# Autodesk Inventor assembly: ARM_042_IntakeFULLAssemblyNewer
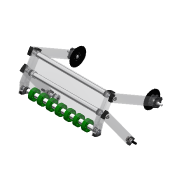
[picture p0: Inventor's stored thumbnail of the model, 180x180]
Saved by Autodesk Inventor 2018 (Build 220112000, 112)
## iProperties
Created: 2020-02-05
Part Number: ARM_042_IntakeFULLAssemblyNewer
Document SubType Name: Assembly
Designer: 22turnmaxw
Mass: 4854.19 g
Surface Area: 17228.7 cm^2
Volume: 2157.03 cm^3
Density: 2.25041 g/cm^3
Author: 22turnmaxw
## Documents named in this file (30)
- C:\Users\Myers.000\Documents\GrabCAD\Infinite Recharge 2020\Build season\ARM_042_IntakeFULLAssemblyNewer.iam
- C:\Users\Myers.000\Documents\GrabCAD\Infinite Recharge 2020\Build season\ARM_031_TwoPieceIntake.iam
- C:\Users\Myers.000\Documents\GrabCAD\Infinite Recharge 2020\Build season\ARM_032_3_OD_Straight_Flex_Wheel_217-6447.ipt
- C:\Users\Myers.000\Documents\GrabCAD\Infinite Recharge 2020\Build season\ARM_036_TopandBottomRollers.iam
- C:\Users\Myers.000\Documents\GrabCAD\Infinite Recharge 2020\Build season\ARM_072_SideBar13v2.ipt
- C:\Users\Myers.000\Documents\GrabCAD\Infinite Recharge 2020\Build season\ARM_071_SideBar15v2.ipt
- C:\Users\Myers.000\Documents\GrabCAD\Infinite Recharge 2020\Build season\ARM_039_MiddleRoller.iam
- C:\Users\Myers.000\Documents\GrabCAD\Infinite Recharge 2020\Build season\ARM_052_0.375ID_FlangedBearing.ipt
- C:\Users\Myers.000\Documents\GrabCAD\Infinite Recharge 2020\Build season\ARM_053_1.5inShoulderScrew.ipt
- C:\Users\Myers.000\Documents\GrabCAD\Infinite Recharge 2020\Build season\ARM_054_0.0625inSpacer.ipt
- C:\Users\Myers.000\Documents\GrabCAD\Infinite Recharge 2020\Build season\ARM_057_1.125inThunderHexBearing.ipt
- C:\Users\Myers.000\Documents\GrabCAD\Infinite Recharge 2020\Build season\ARM_058_BottomRoller.iam
- C:\Users\Myers.000\Documents\GrabCAD\Infinite Recharge 2020\Build season\_64t_Aluminum_Plate_Sprocket_25_Chain_1-1_8_Bearing_Bore_217-2629.ipt
- C:\Users\Myers.000\Documents\GrabCAD\Infinite Recharge 2020\Build season\VersaBlock_V2_217-6111_Combined.iam
- C:\Users\Myers.000\Documents\GrabCAD\Infinite Recharge 2020\Build season\ARM_060_1_125_Bearing_Pilot_Plastic_VersaHub_1_4_Wide_w_Plate_Sprocket_Mount_217-3234.ipt
- C:\Users\Myers.000\Documents\GrabCAD\Infinite Recharge 2020\Build season\ARM_062_4BarDrivingStubAxle.ipt
- C:\Users\Myers.000\Documents\GrabCAD\Infinite Recharge 2020\Build season\ARM_063_IntakeDrivingStubAxle.ipt
- C:\Users\Myers.000\Documents\GrabCAD\Infinite Recharge 2020\Build season\DGB STEP\217-2731_0_500_flanged_bearing.ipt
- C:\Users\Myers.000\Documents\GrabCAD\Infinite Recharge 2020\Build season\ARM_064_Bottom4BarPasiveStubAxle.ipt
- C:\Users\Myers.000\Documents\GrabCAD\Infinite Recharge 2020\Build season\ARM_078_LexanIntakeCover.ipt
- C:\Users\Myers.000\Documents\GrabCAD\Infinite Recharge 2020\Build season\ARM_079_GuiderHolder.ipt
- C:\Users\Myers.000\Documents\GrabCAD\Infinite Recharge 2020\Build season\ARM_077_IntakeBallGuide.ipt
- C:\Users\Myers.000\Documents\GrabCAD\Infinite Recharge 2020\Build season\ARM_083_BallGuideAttachment.ipt
- C:\Users\Myers.000\Documents\GrabCAD\Infinite Recharge 2020\Build season\ARM_082_BallGuideHardstop.ipt
- C:\Users\Myers.000\Documents\GrabCAD\Infinite Recharge 2020\Build season\ARM_034_36Tx9mm3mmPitchPulley.ipt
- C:\Users\Myers.000\Documents\GrabCAD\Infinite Recharge 2020\Build season\ARM_044_SDP_a_6a53-040df0908.ipt
- C:\Users\Myers.000\Documents\GrabCAD\Infinite Recharge 2020\Build season\ARM_084_0.3125Spacer.ipt
- C:\Users\Myers.000\Documents\GrabCAD\Infinite Recharge 2020\Build season\ARM_085_0.0625Spacer.ipt
- C:\Users\Myers.000\Documents\GrabCAD\Infinite Recharge 2020\Build season\ARM_086_1.1875Spacer.ipt
- C:\Users\Myers.000\Documents\GrabCAD\Infinite Recharge 2020\Build season\ARM_091_IntakeSideCap(WithCutout).ipt
## Components (80 placed, 29 different names)
1. ARM_031_TwoPieceIntake:1 [sub-assembly] — Flush:1, Flush:2, Mate:1, Mate:61, Mate:66, Mate:67, Mate:68, Mate:69, Mate:78, Mate:101, Mate:125, Insert:13, Mate:142, Mate:143, Mate:144, Mate:145, Mate:161, Mate:184, Mate:185, Mate:186, Mate:196, Mate:197, Mate:198, Flush:17, Mate:214, Flush:18
2. ARM_031_TwoPieceIntake:2 [sub-assembly] — Flush:1, Flush:2, Mate:1, Mate:63, Mate:64, Mate:65, Mate:70, Mate:73, Mate:74, Mate:76, Mate:77, Mate:83, Mate:84, Mate:91, Mate:92, Mate:110, Mate:111, Mate:113, Mate:114, Mate:115, Insert:6, Mate:187, Mate:188, Mate:189, Mate:199, Mate:200, Mate:201
3. ARM_032_3_OD_Straight_Flex_Wheel_217-6447:1 — Mate:20, Mate:21, Rotation:13, Rotation:14, Mate:155
4. ARM_032_3_OD_Straight_Flex_Wheel_217-6447:2 — Mate:24, Rotation:16, Mate:61, Mate:158
5. ARM_032_3_OD_Straight_Flex_Wheel_217-6447:3 — Mate:22, Mate:23, Mate:24, Rotation:15, Rotation:16, Mate:157
6. ARM_032_3_OD_Straight_Flex_Wheel_217-6447:5 — Mate:18, Rotation:11, Mate:152
7. ARM_032_3_OD_Straight_Flex_Wheel_217-6447:6 — Mate:19, Mate:20, Rotation:12, Rotation:13, Mate:154
8. ARM_032_3_OD_Straight_Flex_Wheel_217-6447:7 — Mate:18, Mate:19, Rotation:11, Rotation:12, Mate:153
9. ARM_032_3_OD_Straight_Flex_Wheel_217-6447:8 — Mate:21, Mate:22, Mate:23, Rotation:14, Rotation:15, Mate:156
10. ARM_036_TopandBottomRollers:2 [sub-assembly] — Mate:76, Mate:78
11. ARM_072_SideBar13v2:1 — Mate:42, Mate:62, Mate:63, Mate:65, Insert:2, Insert:10, Insert:12, Mate:193, Mate:194, Mate:195, Mate:205, Mate:206, Mate:207
12. ARM_072_SideBar13v2:2 — Mate:42, Mate:66, Mate:68, Mate:102, Mate:106, Mate:107, Insert:9, Insert:11, Mate:190, Mate:191, Mate:192, Mate:208, Mate:209, Mate:210
13. ARM_071_SideBar15v2:1 — Mate:43, Mate:60, Mate:64, Mate:70, Mate:85, Mate:86, Mate:129, Mate:131, Mate:132, Angle:1, Mate:202, Mate:203, Mate:204
14. ARM_071_SideBar15v2:2 — Mate:43, Mate:55, Mate:67, Mate:69, Mate:103, Mate:104, Mate:105, Mate:108, Mate:134, Angle:4, Mate:135, Mate:211, Mate:212, Mate:213
15. ARM_039_MiddleRoller:1 [sub-assembly] — Mate:73, Mate:74, Mate:77, Mate:112, Flush:5, Flush:16
16. ARM_052_0.375ID_FlangedBearing:1 — Mate:79, Mate:80, Mate:82, Mate:83, Mate:84
17. ARM_052_0.375ID_FlangedBearing:2 — Mate:81, Mate:82
18. ARM_052_0.375ID_FlangedBearing:3 — Mate:85, Mate:86, Insert:1
19. ARM_052_0.375ID_FlangedBearing:4 — Insert:2, Insert:3
20. ARM_052_0.375ID_FlangedBearing:5 — Mate:87, Mate:88, Mate:90, Mate:91, Mate:92
21. ARM_052_0.375ID_FlangedBearing:6 — Mate:89, Mate:90
22. ARM_052_0.375ID_FlangedBearing:7 — Mate:93, Mate:94, Mate:96
23. ARM_052_0.375ID_FlangedBearing:8 — Mate:95, Mate:96, Mate:103, Mate:104
24. ARM_052_0.375ID_FlangedBearing:9 — Mate:105, Mate:108, Insert:4
25. ARM_052_0.375ID_FlangedBearing:10 — Mate:97, Mate:100
26. ARM_052_0.375ID_FlangedBearing:11 — Mate:106, Mate:107, Insert:5
27. ARM_052_0.375ID_FlangedBearing:12 — Mate:98, Mate:99, Mate:100, Mate:101, Mate:102
28. ARM_053_1.5inShoulderScrew:1 — Insert:4
29. ARM_053_1.5inShoulderScrew:2 — Insert:5
30. ARM_053_1.5inShoulderScrew:3 — Insert:1
31. ARM_053_1.5inShoulderScrew:4 — Insert:3
32. ARM_054_0.0625inSpacer:1 — Mate:79, Mate:80, Mate:81
33. ARM_054_0.0625inSpacer:2 — Mate:87, Mate:88, Mate:89
34. ARM_054_0.0625inSpacer:3 — Mate:93, Mate:94, Mate:95
35. ARM_054_0.0625inSpacer:4 — Mate:97, Mate:98, Mate:99
36. ARM_057_1.125inThunderHexBearing:1 — Mate:110, Mate:111, Mate:116, Mate:117
37. ARM_057_1.125inThunderHexBearing:3 — Mate:114, Mate:115
38. ARM_057_1.125inThunderHexBearing:4 — Mate:112, Mate:113
39. ARM_058_BottomRoller:1 [sub-assembly] — Mate:116, Mate:117, Mate:152, Mate:153, Mate:154, Mate:155, Mate:156, Mate:157, Mate:158
40. ARM_057_1.125inThunderHexBearing:5 — Insert:6
41. ARM_057_1.125inThunderHexBearing:6 — Insert:13
42. ARM_057_1.125inThunderHexBearing:7 — Mate:125, Mate:161
43. _64t_Aluminum_Plate_Sprocket_25_Chain_1-1_8_Bearing_Bore_217-2629:1 — Mate:129, Angle:3, Mate:133, Flush:14
44. VersaBlock_V2_217-6111_Combined:1 [sub-assembly] — Mate:131, Mate:132, Angle:1, Insert:7, Angle:2, Mate:139, Mate:174, Mate:175
45. ARM_060_1_125_Bearing_Pilot_Plastic_VersaHub_1_4_Wide_w_Plate_Sprocket_Mount_217-3234:1 — Insert:7, Angle:2, Angle:3, Mate:133
46. VersaBlock_V2_217-6111_Combined:2 [sub-assembly] — Mate:134, Angle:4, Mate:135, Mate:136, Angle:5, Mate:138, Mate:172, Mate:173, Mate:181
47. ARM_060_1_125_Bearing_Pilot_Plastic_VersaHub_1_4_Wide_w_Plate_Sprocket_Mount_217-3234:2 — Angle:5, Angle:6, Mate:137, Mate:172, Mate:173
48. _64t_Aluminum_Plate_Sprocket_25_Chain_1-1_8_Bearing_Bore_217-2629:2 — Mate:136, Angle:6, Mate:137, Flush:15
49. ARM_062_4BarDrivingStubAxle:1 — Mate:138, Flush:15, Mate:180
50. ARM_062_4BarDrivingStubAxle:2 — Mate:139, Flush:14
51. ARM_063_IntakeDrivingStubAxle:2 — Flush:5, Mate:140, Mate:167
52. 217-2731_0_500_flanged_bearing:1 — Insert:9, Mate:141, Mate:179
53. 217-2731_0_500_flanged_bearing:2 — Insert:11, Flush:6
54. 217-2731_0_500_flanged_bearing:3 — Insert:10, Mate:140, Mate:182
55. 217-2731_0_500_flanged_bearing:4 — Insert:12, Mate:176, Mate:177
56. ARM_064_Bottom4BarPasiveStubAxle:1 — Mate:141, Flush:6, Mate:178
57. ARM_057_1.125inThunderHexBearing:9 — Mate:144, Mate:145
58. ARM_057_1.125inThunderHexBearing:10 — Mate:142, Mate:143
59. ARM_078_LexanIntakeCover:1 — Flush:17, Mate:214, Flush:18, Mate:215
60. ARM_079_GuiderHolder:1 — Mate:160, Flush:10, Mate:163, Mate:164, Mate:215
61. ARM_077_IntakeBallGuide:1 — Mate:160, Flush:10, Mate:162, Flush:11, Flush:12
62. ARM_083_BallGuideAttachment:1 — Mate:162, Flush:11, Flush:12, Flush:13
63. ARM_082_BallGuideHardstop:1 — Mate:163, Flush:13, Mate:164
64. ARM_034_36Tx9mm3mmPitchPulley:1 — Mate:165, Mate:166, Mate:183
65. ARM_044_SDP_a_6a53-040df0908:1 — Mate:165, Mate:166, Flush:16, Mate:167
66. ARM_085_0.0625Spacer:1 — Mate:174, Mate:175
67. ARM_085_0.0625Spacer:2 — Mate:180, Mate:181
68. ARM_084_0.3125Spacer:1 — Mate:176, Mate:177
69. ARM_084_0.3125Spacer:2 — Mate:178, Mate:179
70. ARM_086_1.1875Spacer:1 — Mate:182, Mate:183
71. ARM_091_IntakeSideCap(WithCutout):1 — Mate:184, Mate:185, Mate:186
72. ARM_091_IntakeSideCap(WithCutout):4 — Mate:187, Mate:188, Mate:189
73. ARM_091_IntakeSideCap(WithCutout):6 — Mate:190, Mate:191, Mate:192
74. ARM_091_IntakeSideCap(WithCutout):7 — Mate:193, Mate:194, Mate:195
75. ARM_091_IntakeSideCap(WithCutout):8 — Mate:196, Mate:197, Mate:198
76. ARM_091_IntakeSideCap(WithCutout):9 — Mate:211, Mate:212, Mate:213
77. ARM_091_IntakeSideCap(WithCutout):11 — Mate:199, Mate:200, Mate:201
78. ARM_091_IntakeSideCap(WithCutout):12 — Mate:202, Mate:203, Mate:204
79. ARM_091_IntakeSideCap(WithCutout):14 — Mate:208, Mate:209, Mate:210
80. ARM_091_IntakeSideCap(WithCutout):15 — Mate:205, Mate:206, Mate:207
## Relationships (178: Mate 141, Flush 13, Insert 12, RelateRotation 6, Angle 6)
- Flush:1: ARM_031_TwoPieceIntake:1 ↔ ARM_031_TwoPieceIntake:2
- Flush:2: ARM_031_TwoPieceIntake:1 ↔ ARM_031_TwoPieceIntake:2
- Mate:1 (552.45 mm): ARM_031_TwoPieceIntake:1 ↔ ARM_031_TwoPieceIntake:2
- Mate:18 (44.45 mm): ARM_032_3_OD_Straight_Flex_Wheel_217-6447:5 ↔ ARM_032_3_OD_Straight_Flex_Wheel_217-6447:7
- Mate:19 (44.45 mm): ARM_032_3_OD_Straight_Flex_Wheel_217-6447:6 ↔ ARM_032_3_OD_Straight_Flex_Wheel_217-6447:7
- Mate:20 (44.45 mm): ARM_032_3_OD_Straight_Flex_Wheel_217-6447:1 ↔ ARM_032_3_OD_Straight_Flex_Wheel_217-6447:6
- Mate:21 (44.45 mm): ARM_032_3_OD_Straight_Flex_Wheel_217-6447:1 ↔ ARM_032_3_OD_Straight_Flex_Wheel_217-6447:8
- Mate:22 (44.45 mm): ARM_032_3_OD_Straight_Flex_Wheel_217-6447:3 ↔ ARM_032_3_OD_Straight_Flex_Wheel_217-6447:8
- Mate:23 (44.45 mm): ARM_032_3_OD_Straight_Flex_Wheel_217-6447:3 ↔ ARM_032_3_OD_Straight_Flex_Wheel_217-6447:8
- Mate:24 (44.45 mm): ARM_032_3_OD_Straight_Flex_Wheel_217-6447:2 ↔ ARM_032_3_OD_Straight_Flex_Wheel_217-6447:3
- Rotation:11 [RelateRotation] (1 ul): ARM_032_3_OD_Straight_Flex_Wheel_217-6447:5 ↔ ARM_032_3_OD_Straight_Flex_Wheel_217-6447:7
- Rotation:12 [RelateRotation] (1 ul): ARM_032_3_OD_Straight_Flex_Wheel_217-6447:6 ↔ ARM_032_3_OD_Straight_Flex_Wheel_217-6447:7
- Rotation:13 [RelateRotation] (1 ul): ARM_032_3_OD_Straight_Flex_Wheel_217-6447:1 ↔ ARM_032_3_OD_Straight_Flex_Wheel_217-6447:6
- Rotation:14 [RelateRotation] (1 ul): ARM_032_3_OD_Straight_Flex_Wheel_217-6447:1 ↔ ARM_032_3_OD_Straight_Flex_Wheel_217-6447:8
- Rotation:15 [RelateRotation] (1 ul): ARM_032_3_OD_Straight_Flex_Wheel_217-6447:3 ↔ ARM_032_3_OD_Straight_Flex_Wheel_217-6447:8
- Rotation:16 [RelateRotation] (1 ul): ARM_032_3_OD_Straight_Flex_Wheel_217-6447:2 ↔ ARM_032_3_OD_Straight_Flex_Wheel_217-6447:3
- Mate:42: ARM_072_SideBar13v2:1 ↔ ARM_072_SideBar13v2:2
- Mate:43: ARM_071_SideBar15v2:1 ↔ ARM_071_SideBar15v2:2
- Mate:55 (135.8138 mm): ARM_071_SideBar15v2:2
- Mate:60 (124.4092 mm): ARM_071_SideBar15v2:1
- Mate:61 (50.8 mm): ARM_031_TwoPieceIntake:1 ↔ ARM_032_3_OD_Straight_Flex_Wheel_217-6447:2
- Mate:62: ARM_072_SideBar13v2:1
- Mate:63 (4.7625 mm): ARM_031_TwoPieceIntake:2 ↔ ARM_072_SideBar13v2:1
- Mate:64: ARM_031_TwoPieceIntake:2 ↔ ARM_071_SideBar15v2:1
- Mate:65: ARM_031_TwoPieceIntake:2 ↔ ARM_072_SideBar13v2:1
- Mate:66: ARM_031_TwoPieceIntake:1 ↔ ARM_072_SideBar13v2:2
- Mate:67: ARM_031_TwoPieceIntake:1 ↔ ARM_071_SideBar15v2:2
- Mate:68 (4.7625 mm): ARM_031_TwoPieceIntake:1 ↔ ARM_072_SideBar13v2:2
- Mate:69 (4.7625 mm): ARM_031_TwoPieceIntake:1 ↔ ARM_071_SideBar15v2:2
- Mate:70 (4.7625 mm): ARM_031_TwoPieceIntake:2 ↔ ARM_071_SideBar15v2:1
- Mate:73: ARM_031_TwoPieceIntake:2 ↔ ARM_039_MiddleRoller:1
- Mate:74: ARM_031_TwoPieceIntake:2 ↔ ARM_039_MiddleRoller:1
- Mate:76: ARM_031_TwoPieceIntake:2 ↔ ARM_036_TopandBottomRollers:2
- Mate:77 (1.5875 mm): ARM_031_TwoPieceIntake:2 ↔ ARM_039_MiddleRoller:1
- Mate:78 (1.5875 mm): ARM_031_TwoPieceIntake:1 ↔ ARM_036_TopandBottomRollers:2
- Mate:79: ARM_052_0.375ID_FlangedBearing:1 ↔ ARM_054_0.0625inSpacer:1
- Mate:80: ARM_052_0.375ID_FlangedBearing:1 ↔ ARM_054_0.0625inSpacer:1
- Mate:81: ARM_052_0.375ID_FlangedBearing:2 ↔ ARM_054_0.0625inSpacer:1
- Mate:82: ARM_052_0.375ID_FlangedBearing:1 ↔ ARM_052_0.375ID_FlangedBearing:2
- Mate:83: ARM_031_TwoPieceIntake:2 ↔ ARM_052_0.375ID_FlangedBearing:1
- Mate:84: ARM_031_TwoPieceIntake:2 ↔ ARM_052_0.375ID_FlangedBearing:1
- Mate:85: ARM_071_SideBar15v2:1 ↔ ARM_052_0.375ID_FlangedBearing:3
- Mate:86: ARM_071_SideBar15v2:1 ↔ ARM_052_0.375ID_FlangedBearing:3
- Insert:1: ARM_052_0.375ID_FlangedBearing:3 ↔ ARM_053_1.5inShoulderScrew:3
- Mate:87: ARM_052_0.375ID_FlangedBearing:5 ↔ ARM_054_0.0625inSpacer:2
- Mate:88: ARM_052_0.375ID_FlangedBearing:5 ↔ ARM_054_0.0625inSpacer:2
- Mate:89: ARM_052_0.375ID_FlangedBearing:6 ↔ ARM_054_0.0625inSpacer:2
- Mate:90: ARM_052_0.375ID_FlangedBearing:5 ↔ ARM_052_0.375ID_FlangedBearing:6
- Mate:91: ARM_031_TwoPieceIntake:2 ↔ ARM_052_0.375ID_FlangedBearing:5
- Mate:92: ARM_031_TwoPieceIntake:2 ↔ ARM_052_0.375ID_FlangedBearing:5
- Insert:2: ARM_072_SideBar13v2:1 ↔ ARM_052_0.375ID_FlangedBearing:4
- Insert:3: ARM_052_0.375ID_FlangedBearing:4 ↔ ARM_053_1.5inShoulderScrew:4
- Mate:93: ARM_052_0.375ID_FlangedBearing:7 ↔ ARM_054_0.0625inSpacer:3
- Mate:94: ARM_052_0.375ID_FlangedBearing:7 ↔ ARM_054_0.0625inSpacer:3
- Mate:95: ARM_052_0.375ID_FlangedBearing:8 ↔ ARM_054_0.0625inSpacer:3
- Mate:96: ARM_052_0.375ID_FlangedBearing:7 ↔ ARM_052_0.375ID_FlangedBearing:8
- Mate:97: ARM_052_0.375ID_FlangedBearing:10 ↔ ARM_054_0.0625inSpacer:4
- Mate:98: ARM_052_0.375ID_FlangedBearing:12 ↔ ARM_054_0.0625inSpacer:4
- Mate:99: ARM_052_0.375ID_FlangedBearing:12 ↔ ARM_054_0.0625inSpacer:4
- Mate:100: ARM_052_0.375ID_FlangedBearing:10 ↔ ARM_052_0.375ID_FlangedBearing:12
- Mate:101: ARM_031_TwoPieceIntake:1 ↔ ARM_052_0.375ID_FlangedBearing:12
- Mate:102: ARM_072_SideBar13v2:2 ↔ ARM_052_0.375ID_FlangedBearing:12
- Mate:103: ARM_071_SideBar15v2:2 ↔ ARM_052_0.375ID_FlangedBearing:8
- Mate:104: ARM_071_SideBar15v2:2 ↔ ARM_052_0.375ID_FlangedBearing:8
- Mate:105: ARM_071_SideBar15v2:2 ↔ ARM_052_0.375ID_FlangedBearing:9
- Mate:106: ARM_072_SideBar13v2:2 ↔ ARM_052_0.375ID_FlangedBearing:11
- Mate:107: ARM_072_SideBar13v2:2 ↔ ARM_052_0.375ID_FlangedBearing:11
- Mate:108: ARM_071_SideBar15v2:2 ↔ ARM_052_0.375ID_FlangedBearing:9
- Insert:4: ARM_052_0.375ID_FlangedBearing:9 ↔ ARM_053_1.5inShoulderScrew:1
- Insert:5: ARM_052_0.375ID_FlangedBearing:11 ↔ ARM_053_1.5inShoulderScrew:2
- Mate:110: ARM_031_TwoPieceIntake:2 ↔ ARM_057_1.125inThunderHexBearing:1
- Mate:111: ARM_031_TwoPieceIntake:2 ↔ ARM_057_1.125inThunderHexBearing:1
- Mate:112: ARM_039_MiddleRoller:1 ↔ ARM_057_1.125inThunderHexBearing:4
- Mate:113: ARM_031_TwoPieceIntake:2 ↔ ARM_057_1.125inThunderHexBearing:4
- Mate:114: ARM_031_TwoPieceIntake:2 ↔ ARM_057_1.125inThunderHexBearing:3
- Mate:115: ARM_031_TwoPieceIntake:2 ↔ ARM_057_1.125inThunderHexBearing:3
- Mate:116: ARM_057_1.125inThunderHexBearing:1 ↔ ARM_058_BottomRoller:1
- Mate:117: ARM_057_1.125inThunderHexBearing:1 ↔ ARM_058_BottomRoller:1
- Insert:6: ARM_031_TwoPieceIntake:2 ↔ ARM_057_1.125inThunderHexBearing:5
- Mate:125: ARM_031_TwoPieceIntake:1 ↔ ARM_057_1.125inThunderHexBearing:7
- Mate:129: ARM_071_SideBar15v2:1 ↔ _64t_Aluminum_Plate_Sprocket_25_Chain_1-1_8_Bearing_Bore_217-2629:1
- Mate:131: ARM_071_SideBar15v2:1 ↔ VersaBlock_V2_217-6111_Combined:1
- Mate:132: ARM_071_SideBar15v2:1 ↔ VersaBlock_V2_217-6111_Combined:1
- Angle:1 (0 deg): ARM_071_SideBar15v2:1 ↔ VersaBlock_V2_217-6111_Combined:1
- Insert:7: VersaBlock_V2_217-6111_Combined:1 ↔ ARM_060_1_125_Bearing_Pilot_Plastic_VersaHub_1_4_Wide_w_Plate_Sprocket_Mount_217-3234:1
- Angle:2 (0 deg): VersaBlock_V2_217-6111_Combined:1 ↔ ARM_060_1_125_Bearing_Pilot_Plastic_VersaHub_1_4_Wide_w_Plate_Sprocket_Mount_217-3234:1
- Angle:3 (0 deg): _64t_Aluminum_Plate_Sprocket_25_Chain_1-1_8_Bearing_Bore_217-2629:1 ↔ ARM_060_1_125_Bearing_Pilot_Plastic_VersaHub_1_4_Wide_w_Plate_Sprocket_Mount_217-3234:1
- Mate:133: _64t_Aluminum_Plate_Sprocket_25_Chain_1-1_8_Bearing_Bore_217-2629:1 ↔ ARM_060_1_125_Bearing_Pilot_Plastic_VersaHub_1_4_Wide_w_Plate_Sprocket_Mount_217-3234:1
- Mate:134: ARM_071_SideBar15v2:2 ↔ VersaBlock_V2_217-6111_Combined:2
- Angle:4 (0 deg): ARM_071_SideBar15v2:2 ↔ VersaBlock_V2_217-6111_Combined:2
- Mate:135: ARM_071_SideBar15v2:2 ↔ VersaBlock_V2_217-6111_Combined:2
- Mate:136: VersaBlock_V2_217-6111_Combined:2 ↔ _64t_Aluminum_Plate_Sprocket_25_Chain_1-1_8_Bearing_Bore_217-2629:2
- Angle:5 (0 deg): VersaBlock_V2_217-6111_Combined:2 ↔ ARM_060_1_125_Bearing_Pilot_Plastic_VersaHub_1_4_Wide_w_Plate_Sprocket_Mount_217-3234:2
- Angle:6 (0 deg): ARM_060_1_125_Bearing_Pilot_Plastic_VersaHub_1_4_Wide_w_Plate_Sprocket_Mount_217-3234:2 ↔ _64t_Aluminum_Plate_Sprocket_25_Chain_1-1_8_Bearing_Bore_217-2629:2
- Mate:137: ARM_060_1_125_Bearing_Pilot_Plastic_VersaHub_1_4_Wide_w_Plate_Sprocket_Mount_217-3234:2 ↔ _64t_Aluminum_Plate_Sprocket_25_Chain_1-1_8_Bearing_Bore_217-2629:2
- Mate:138: VersaBlock_V2_217-6111_Combined:2 ↔ ARM_062_4BarDrivingStubAxle:1
- Mate:139: VersaBlock_V2_217-6111_Combined:1 ↔ ARM_062_4BarDrivingStubAxle:2
- Insert:9: ARM_072_SideBar13v2:2 ↔ 217-2731_0_500_flanged_bearing:1
- Insert:10: ARM_072_SideBar13v2:1 ↔ 217-2731_0_500_flanged_bearing:3
- Insert:11: ARM_072_SideBar13v2:2 ↔ 217-2731_0_500_flanged_bearing:2
- Insert:12: ARM_072_SideBar13v2:1 ↔ 217-2731_0_500_flanged_bearing:4
- Insert:13: ARM_031_TwoPieceIntake:1 ↔ ARM_057_1.125inThunderHexBearing:6
- Flush:5: ARM_039_MiddleRoller:1 ↔ ARM_063_IntakeDrivingStubAxle:2
- Mate:140: ARM_063_IntakeDrivingStubAxle:2 ↔ 217-2731_0_500_flanged_bearing:3
- Mate:141: 217-2731_0_500_flanged_bearing:1 ↔ ARM_064_Bottom4BarPasiveStubAxle:1
- Flush:6: 217-2731_0_500_flanged_bearing:2 ↔ ARM_064_Bottom4BarPasiveStubAxle:1
- Mate:142: ARM_031_TwoPieceIntake:1 ↔ ARM_057_1.125inThunderHexBearing:10
- Mate:143: ARM_031_TwoPieceIntake:1 ↔ ARM_057_1.125inThunderHexBearing:10
- Mate:144: ARM_031_TwoPieceIntake:1 ↔ ARM_057_1.125inThunderHexBearing:9
- Mate:145: ARM_031_TwoPieceIntake:1 ↔ ARM_057_1.125inThunderHexBearing:9
- Mate:152: ARM_032_3_OD_Straight_Flex_Wheel_217-6447:5 ↔ ARM_058_BottomRoller:1
- Mate:153: ARM_032_3_OD_Straight_Flex_Wheel_217-6447:7 ↔ ARM_058_BottomRoller:1
- Mate:154: ARM_032_3_OD_Straight_Flex_Wheel_217-6447:6 ↔ ARM_058_BottomRoller:1
- Mate:155: ARM_032_3_OD_Straight_Flex_Wheel_217-6447:1 ↔ ARM_058_BottomRoller:1
- Mate:156: ARM_032_3_OD_Straight_Flex_Wheel_217-6447:8 ↔ ARM_058_BottomRoller:1
- Mate:157: ARM_032_3_OD_Straight_Flex_Wheel_217-6447:3 ↔ ARM_058_BottomRoller:1
- Mate:158: ARM_032_3_OD_Straight_Flex_Wheel_217-6447:2 ↔ ARM_058_BottomRoller:1
- Mate:160: ARM_079_GuiderHolder:1 ↔ ARM_077_IntakeBallGuide:1
- Flush:10 (158.75 mm): ARM_079_GuiderHolder:1 ↔ ARM_077_IntakeBallGuide:1
- Mate:161: ARM_031_TwoPieceIntake:1 ↔ ARM_057_1.125inThunderHexBearing:7
- Mate:162: ARM_077_IntakeBallGuide:1 ↔ ARM_083_BallGuideAttachment:1
- Flush:11 (-12.7 mm): ARM_077_IntakeBallGuide:1 ↔ ARM_083_BallGuideAttachment:1
- Flush:12 (-127 mm): ARM_077_IntakeBallGuide:1 ↔ ARM_083_BallGuideAttachment:1
- Mate:163: ARM_079_GuiderHolder:1 ↔ ARM_082_BallGuideHardstop:1
- Flush:13: ARM_083_BallGuideAttachment:1 ↔ ARM_082_BallGuideHardstop:1
- Mate:164 (-24.8412 mm): ARM_079_GuiderHolder:1 ↔ ARM_082_BallGuideHardstop:1
- Flush:14: _64t_Aluminum_Plate_Sprocket_25_Chain_1-1_8_Bearing_Bore_217-2629:1 ↔ ARM_062_4BarDrivingStubAxle:2
- Flush:15: _64t_Aluminum_Plate_Sprocket_25_Chain_1-1_8_Bearing_Bore_217-2629:2 ↔ ARM_062_4BarDrivingStubAxle:1
- Mate:165: ARM_034_36Tx9mm3mmPitchPulley:1 ↔ ARM_044_SDP_a_6a53-040df0908:1
- Mate:166: ARM_034_36Tx9mm3mmPitchPulley:1 ↔ ARM_044_SDP_a_6a53-040df0908:1
- Flush:16: ARM_039_MiddleRoller:1 ↔ ARM_044_SDP_a_6a53-040df0908:1
- Mate:167: ARM_063_IntakeDrivingStubAxle:2 ↔ ARM_044_SDP_a_6a53-040df0908:1
- Mate:172: VersaBlock_V2_217-6111_Combined:2 ↔ ARM_060_1_125_Bearing_Pilot_Plastic_VersaHub_1_4_Wide_w_Plate_Sprocket_Mount_217-3234:2
- Mate:173: VersaBlock_V2_217-6111_Combined:2 ↔ ARM_060_1_125_Bearing_Pilot_Plastic_VersaHub_1_4_Wide_w_Plate_Sprocket_Mount_217-3234:2
- Mate:174: VersaBlock_V2_217-6111_Combined:1 ↔ ARM_085_0.0625Spacer:1
- Mate:175: VersaBlock_V2_217-6111_Combined:1 ↔ ARM_085_0.0625Spacer:1
- Mate:176: 217-2731_0_500_flanged_bearing:4 ↔ ARM_084_0.3125Spacer:1
- Mate:177: 217-2731_0_500_flanged_bearing:4 ↔ ARM_084_0.3125Spacer:1
- Mate:178: ARM_064_Bottom4BarPasiveStubAxle:1 ↔ ARM_084_0.3125Spacer:2
- Mate:179: 217-2731_0_500_flanged_bearing:1 ↔ ARM_084_0.3125Spacer:2
- Mate:180: ARM_062_4BarDrivingStubAxle:1 ↔ ARM_085_0.0625Spacer:2
- Mate:181: VersaBlock_V2_217-6111_Combined:2 ↔ ARM_085_0.0625Spacer:2
- Mate:182: 217-2731_0_500_flanged_bearing:3 ↔ ARM_086_1.1875Spacer:1
- Mate:183: ARM_034_36Tx9mm3mmPitchPulley:1 ↔ ARM_086_1.1875Spacer:1
- Mate:184: ARM_031_TwoPieceIntake:1 ↔ ARM_091_IntakeSideCap(WithCutout):1
- Mate:185: ARM_031_TwoPieceIntake:1 ↔ ARM_091_IntakeSideCap(WithCutout):1
- Mate:186: ARM_031_TwoPieceIntake:1 ↔ ARM_091_IntakeSideCap(WithCutout):1
- Mate:187: ARM_031_TwoPieceIntake:2 ↔ ARM_091_IntakeSideCap(WithCutout):4
- Mate:188: ARM_031_TwoPieceIntake:2 ↔ ARM_091_IntakeSideCap(WithCutout):4
- Mate:189: ARM_031_TwoPieceIntake:2 ↔ ARM_091_IntakeSideCap(WithCutout):4
- Mate:190: ARM_072_SideBar13v2:2 ↔ ARM_091_IntakeSideCap(WithCutout):6
- Mate:191: ARM_072_SideBar13v2:2 ↔ ARM_091_IntakeSideCap(WithCutout):6
- Mate:192: ARM_072_SideBar13v2:2 ↔ ARM_091_IntakeSideCap(WithCutout):6
- Mate:193: ARM_072_SideBar13v2:1 ↔ ARM_091_IntakeSideCap(WithCutout):7
- Mate:194: ARM_072_SideBar13v2:1 ↔ ARM_091_IntakeSideCap(WithCutout):7
- Mate:195: ARM_072_SideBar13v2:1 ↔ ARM_091_IntakeSideCap(WithCutout):7
- Mate:196: ARM_031_TwoPieceIntake:1 ↔ ARM_091_IntakeSideCap(WithCutout):8
- Mate:197: ARM_031_TwoPieceIntake:1 ↔ ARM_091_IntakeSideCap(WithCutout):8
- Mate:198: ARM_031_TwoPieceIntake:1 ↔ ARM_091_IntakeSideCap(WithCutout):8
- Mate:199: ARM_031_TwoPieceIntake:2 ↔ ARM_091_IntakeSideCap(WithCutout):11
- Mate:200: ARM_031_TwoPieceIntake:2 ↔ ARM_091_IntakeSideCap(WithCutout):11
- Mate:201: ARM_031_TwoPieceIntake:2 ↔ ARM_091_IntakeSideCap(WithCutout):11
- Mate:202: ARM_071_SideBar15v2:1 ↔ ARM_091_IntakeSideCap(WithCutout):12
- Mate:203: ARM_071_SideBar15v2:1 ↔ ARM_091_IntakeSideCap(WithCutout):12
- Mate:204: ARM_071_SideBar15v2:1 ↔ ARM_091_IntakeSideCap(WithCutout):12
- Mate:205: ARM_072_SideBar13v2:1 ↔ ARM_091_IntakeSideCap(WithCutout):15
- Mate:206: ARM_072_SideBar13v2:1 ↔ ARM_091_IntakeSideCap(WithCutout):15
- Mate:207: ARM_072_SideBar13v2:1 ↔ ARM_091_IntakeSideCap(WithCutout):15
- Mate:208: ARM_072_SideBar13v2:2 ↔ ARM_091_IntakeSideCap(WithCutout):14
- Mate:209: ARM_072_SideBar13v2:2 ↔ ARM_091_IntakeSideCap(WithCutout):14
- Mate:210: ARM_072_SideBar13v2:2 ↔ ARM_091_IntakeSideCap(WithCutout):14
- Mate:211: ARM_071_SideBar15v2:2 ↔ ARM_091_IntakeSideCap(WithCutout):9
- Mate:212: ARM_071_SideBar15v2:2 ↔ ARM_091_IntakeSideCap(WithCutout):9
- Mate:213: ARM_071_SideBar15v2:2 ↔ ARM_091_IntakeSideCap(WithCutout):9
- Flush:17: ARM_031_TwoPieceIntake:1 ↔ ARM_078_LexanIntakeCover:1
- Mate:214: ARM_031_TwoPieceIntake:1 ↔ ARM_078_LexanIntakeCover:1
- Flush:18: ARM_031_TwoPieceIntake:1 ↔ ARM_078_LexanIntakeCover:1
- Mate:215: ARM_078_LexanIntakeCover:1 ↔ ARM_079_GuiderHolder:1
